# Autodesk Inventor assembly: Display_Unit
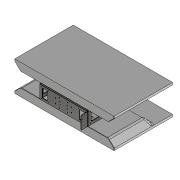
[picture p0: Inventor's stored thumbnail of the model, 180x180]
Saved by Autodesk Inventor 2020 (Build 240168000, 168)
## iProperties
Created: 2021-12-05
Part Number: Display_Unit
Document SubType Name: Assembly
Designer: ken113
Mass: 17421.3 g
Surface Area: 19459.9 cm^2
Volume: 27621.8 cm^3
Density: 0.630708 g/cm^3
Author: ken113
## Documents named in this file (5)
- D:\Documents\GitHub\Eto_Project\Hardware\Asem\Display_Unit.iam
- D:\Documents\GitHub\Eto_Project\Hardware\Parts\Display\Display_B.ipt
- D:\Documents\GitHub\Eto_Project\Hardware\Parts\Meviy\New_Meviy\Display_Mount_A.ipt
- D:\Documents\GitHub\Eto_Project\Hardware\Parts\Meviy\New_Meviy\Display_Mount_B.ipt
- D:\Documents\GitHub\Eto_Project\Hardware\Parts\Grabcad\raspberry-pi-4-model-b-03-1.snapshot.1\Raspberry-Pi-4-Model-B-03.ipt
## Components (5 placed, 4 different names)
1. Display_B:1 — メイト:1, メイト:2, 挿入:1, 挿入:2
2. Display_B:2 — メイト:1, メイト:2, 挿入:3, 挿入:4
3. Display_Mount_A:1 — 挿入:1, 挿入:2, メイト:3
4. Display_Mount_B:1 — 挿入:3, 挿入:4, メイト:3, メイト:4, 角度:1
5. Raspberry-Pi-4-Model-B-03:1 — メイト:4, 角度:1
## Relationships (9: Mate 4, Insert 4, Angle 1)
- メイト:1 [Mate]: Display_B:1 ↔ Display_B:2
- メイト:2 [Mate]: Display_B:1 ↔ Display_B:2
- 挿入:1 [Insert]: Display_B:1 ↔ Display_Mount_A:1
- 挿入:2 [Insert]: Display_B:1 ↔ Display_Mount_A:1
- 挿入:3 [Insert]: Display_B:2 ↔ Display_Mount_B:1
- 挿入:4 [Insert]: Display_B:2 ↔ Display_Mount_B:1
- メイト:3 [Mate]: Display_Mount_A:1 ↔ Display_Mount_B:1
- メイト:4 [Mate] (10 mm): Display_Mount_B:1 ↔ Raspberry-Pi-4-Model-B-03:1
- 角度:1 [Angle] (0 deg): Display_Mount_B:1 ↔ Raspberry-Pi-4-Model-B-03:1
